# Autodesk Inventor assembly: ASY Beshkino_bio_tank
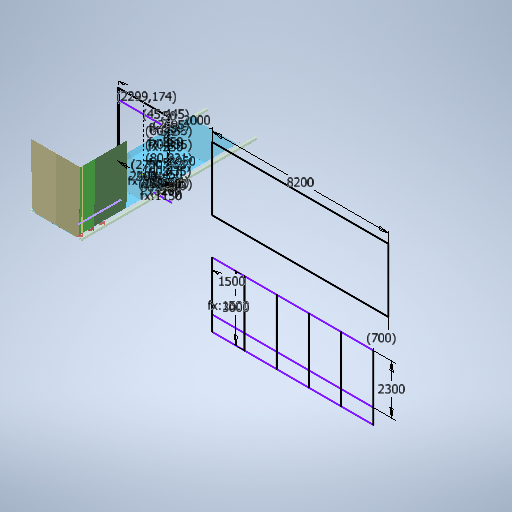
[picture p0: Inventor's stored thumbnail of the model, 512x512]
Saved by Autodesk Inventor 2025 (Build 290162010, 162A)
## iProperties
Created: 2024-07-21
Part Number: ASY Beshkino_bio_tank
Document SubType Name: Assembly
Designer: admin
Author: admin
## Documents named in this file (10)
- C:\Users\admin\YandexDisk-badmisterfox\домашниий пк\Inventor\BSH_Beshkino_bio_tank\ASY Beshkino_bio_tank.iam
- C:\Users\admin\YandexDisk-badmisterfox\домашниий пк\Inventor\BSH_Beshkino_bio_tank\BSH 000 dim Beshkino_bio_tank.ipt
- C:\Users\admin\YandexDisk-badmisterfox\домашниий пк\Inventor\BSH_Beshkino_bio_tank\BSH 010 floor 1.ipt
- C:\Users\admin\YandexDisk-badmisterfox\домашниий пк\Inventor\BSH_Beshkino_bio_tank\BSH 021 rib 1.ipt
- C:\Users\admin\YandexDisk-badmisterfox\домашниий пк\Inventor\BSH_Beshkino_bio_tank\BSH 022 rib 2.ipt
- C:\Users\admin\YandexDisk-badmisterfox\домашниий пк\Inventor\BSH_Beshkino_bio_tank\BSH 061 tube 1.ipt
- C:\Users\admin\YandexDisk-badmisterfox\домашниий пк\Inventor\BSH_Beshkino_bio_tank\BSH 031 nose 1.ipt
- C:\Users\admin\YandexDisk-badmisterfox\домашниий пк\Inventor\BSH_Beshkino_bio_tank\BSH 032 board 2.ipt
- C:\Users\admin\YandexDisk-badmisterfox\домашниий пк\Inventor\BSH_Beshkino_bio_tank\BSH 033 board 3.ipt
- C:\Users\admin\YandexDisk-badmisterfox\домашниий пк\Inventor\BSH_Beshkino_bio_tank\BSH 041 stringer 1.ipt
## Components (18 placed, 9 different names)
1. BSH 000 dim Beshkino_bio_tank:1
2. BSH 010 floor 1:1 — Mate:5, Mate:6, Rigid:4, Mate:7, Flush:4, Mate:10, Flush:5
3. BSH 020 rib 1:1 — Mate:4, Flush:3, Mate:5, Mate:6, Rigid:2, Rigid:3, Rigid:9
4. BSH 022 rib 2:1 — Rigid:3, Mate:8, Rigid:12
5. BSH 061 tube 1:1 — Mate:1, Rigid:1, Mate:3
6. BSH 061 tube 1:2 — Mate:2, Rigid:1, Mate:4, Flush:3, Flush:4
7. BSH 020 rib 1:2 — Rigid:2
8. BSH 031 nose 1:1 — Mate:10, Flush:5, Mate:11, Rigid:11
9. BSH 010 floor 1:2 — Rigid:4, Rigid:5
10. BSH 010 floor 1:3 — Rigid:5, Rigid:6, Mate:9
11. BSH 010 floor 1:4 — Rigid:6, Rigid:7
12. BSH 010 floor 1:5 — Rigid:7
13. BSH 032 board 2:1 — Mate:8, Mate:9, Rigid:8
14. BSH 033 board 3:1 — Rigid:8
15. BSH 020 rib 1:3 — Rigid:9, Rigid:10
16. BSH 020 rib 1:4 — Rigid:10
17. BSH 031 nose 1:2 — Rigid:11
18. BSH 041 stringer 1:1 — Rigid:12
## Relationships (26: WeldJoint 12, Mate 11, Flush 3)
- Mate:1: BSH 061 tube 1:1
- Mate:2: BSH 061 tube 1:2
- Rigid:1 [WeldJoint] (-2400 mm): BSH 061 tube 1:1 ↔ BSH 061 tube 1:2
- Mate:3: BSH 061 tube 1:1
- Mate:4: BSH 020 rib 1:1 ↔ BSH 061 tube 1:2
- Flush:3: BSH 020 rib 1:1 ↔ BSH 061 tube 1:2
- Mate:5: BSH 010 floor 1:1 ↔ BSH 020 rib 1:1
- Mate:6: BSH 010 floor 1:1 ↔ BSH 020 rib 1:1
- Rigid:2 [WeldJoint]: BSH 020 rib 1:1 ↔ BSH 020 rib 1:2
- Rigid:3 [WeldJoint]: BSH 020 rib 1:1 ↔ BSH 022 rib 2:1
- Rigid:4 [WeldJoint]: BSH 010 floor 1:1 ↔ BSH 010 floor 1:2
- Rigid:5 [WeldJoint]: BSH 010 floor 1:2 ↔ BSH 010 floor 1:3
- Rigid:6 [WeldJoint]: BSH 010 floor 1:3 ↔ BSH 010 floor 1:4
- Rigid:7 [WeldJoint]: BSH 010 floor 1:4 ↔ BSH 010 floor 1:5
- Mate:7: BSH 010 floor 1:1
- Flush:4: BSH 010 floor 1:1 ↔ BSH 061 tube 1:2
- Mate:8: BSH 022 rib 2:1 ↔ BSH 032 board 2:1
- Mate:9: BSH 010 floor 1:3 ↔ BSH 032 board 2:1
- Rigid:8 [WeldJoint]: BSH 032 board 2:1 ↔ BSH 033 board 3:1
- Rigid:9 [WeldJoint] (-500 mm): BSH 020 rib 1:1 ↔ BSH 020 rib 1:3
- Rigid:10 [WeldJoint] (-500 mm): BSH 020 rib 1:3 ↔ BSH 020 rib 1:4
- Mate:10: BSH 010 floor 1:1 ↔ BSH 031 nose 1:1
- Flush:5 (10 mm): BSH 010 floor 1:1 ↔ BSH 031 nose 1:1
- Mate:11: BSH 031 nose 1:1
- Rigid:11 [WeldJoint]: BSH 031 nose 1:1 ↔ BSH 031 nose 1:2
- Rigid:12 [WeldJoint] (2 mm): BSH 022 rib 2:1 ↔ BSH 041 stringer 1:1
